# Autodesk Inventor assembly: FRAMEBOX
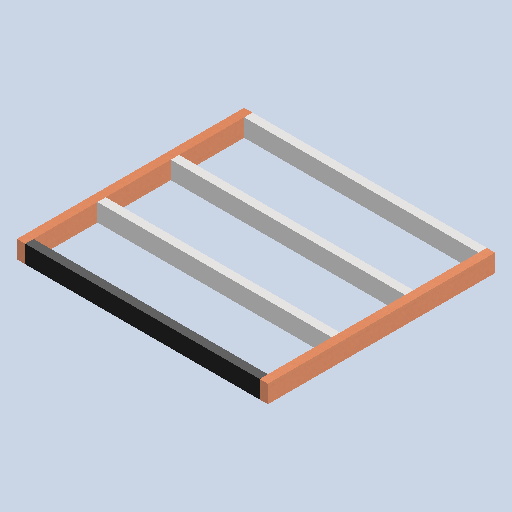
[picture p0: Inventor's stored thumbnail of the model, 512x512]
Saved by Autodesk Inventor 2023 (Build 270158000, 158)
## iProperties
Created: 2022-07-13
Part Number: FRAMEBOX
Document SubType Name: Assembly
Designer: plebbb
Author: plebbb
## Documents named in this file (3)
- D:\Users\plebbb\Desktop\CNC_Project\WOOD\FRAMEBOX.iam
- D:\Users\plebbb\Desktop\CNC_Project\WOOD\2x4x48.ipt
- D:\Users\plebbb\Desktop\CNC_Project\WOOD\2x4x49.5.ipt
## Components (6 placed, 2 different names)
1. 2x4x48:1
2. 2x4x48:2
3. 2x4x49.5:1
4. 2x4x49.5:2
5. 2x4x49.5:3
6. 2x4x49.5:4
## Component patterns: (3 elements, first: 2x4x49.5:2)
## Relationships (4: Mate 2, Flush 2)
- [Mate]: 2x4x48:2 ↔ 2x4x49.5:1
- [Flush]: 2x4x48:1 ↔ 2x4x49.5:1
- [Flush]: 2x4x48:1 ↔ 2x4x49.5:2
- [Mate]: 2x4x48:2 ↔ 2x4x49.5:2
